# Autodesk Inventor assembly: PS20021
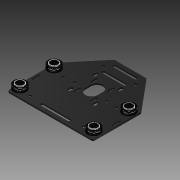
[picture p0: Inventor's stored thumbnail of the model, 180x180]
Saved by Autodesk Inventor 2014 (Build 180170000, 170)
## iProperties
Created: 2013-05-29
Part Number: PS20021
Document SubType Name: Assembly
Designer: Edward
Description: Z-Assembly Carriage
Author: Edward
Title: Z-Assembly Carriage
Subject: Shapeoko 2
## Documents named in this file (7)
- C:\Users\Edward\Documents\GitHub\Shapeoko_2\Autodesk_Inventor_Project\PS20021.iam
- C:\Users\Edward\Documents\GitHub\Shapeoko_2\Autodesk_Inventor_Project\26029-01.ipt
- C:\Users\Edward\Documents\GitHub\Shapeoko_2\Autodesk_Inventor_Project\30158-01.ipt
- C:\Users\Edward\Documents\GitHub\Shapeoko_2\Autodesk_Inventor_Project\25203-02.iam
- C:\Users\Edward\Documents\GitHub\Shapeoko_2\Autodesk_Inventor_Project\PS20004.ipt
- C:\Users\Edward\Documents\GitHub\Shapeoko_2\Autodesk_Inventor_Project\25287-02.ipt
- C:\Users\Edward\Documents\GitHub\Shapeoko_2\Autodesk_Inventor_Project\25284-02.ipt
## Components (19 placed, 6 different names)
1. 26029-01:1 — Insert:3, Insert:5, Insert:9, Mate:2, Insert:10, Mate:4, Insert:15, Insert:16
2. 30158-01:1 — Insert:10, Mate:3
3. 30158-01:2 — Mate:1, Insert:9
4. 25203-02:4 [sub-assembly] — Insert:2, Insert:4
5. 25287-02:1 — Insert:2, Insert:3
6. PS20004:2 — Insert:4
7. 25287-02:2 — Insert:11, Mate:4
8. 25284-02:2 — Insert:6
9. 25287-02:4 — Insert:16, Insert:17
10. 25287-02:5 — Insert:14, Insert:15
11. 25287-02:6 — Insert:7, Mate:2
12. 25287-02:7 — Insert:5, Insert:6
13. PS20004:3 — Insert:8, Mate:1
14. 25203-02:5 [sub-assembly] — Insert:7, Insert:8
15. PS20004:4 — Insert:12, Mate:3
16. 25203-02:6 [sub-assembly] — Insert:11, Insert:12
17. PS20004:5 — Insert:13
18. 25203-02:7 [sub-assembly] — Insert:13, Insert:14
19. 25284-02:3 — Insert:17
## Relationships (20: Insert 16, Mate 4)
- Insert:2: 25203-02:4 ↔ 25287-02:1
- Insert:3: 26029-01:1 ↔ 25287-02:1
- Insert:4: 25203-02:4 ↔ PS20004:2
- Insert:5: 26029-01:1 ↔ 25287-02:7
- Insert:6: 25284-02:2 ↔ 25287-02:7
- Insert:7: 25287-02:6 ↔ 25203-02:5
- Insert:8: PS20004:3 ↔ 25203-02:5
- Mate:1: 30158-01:2 ↔ PS20004:3
- Insert:9: 26029-01:1 ↔ 30158-01:2
- Mate:2: 26029-01:1 ↔ 25287-02:6
- Insert:10: 26029-01:1 ↔ 30158-01:1
- Insert:11: 25287-02:2 ↔ 25203-02:6
- Insert:12: PS20004:4 ↔ 25203-02:6
- Mate:3: 30158-01:1 ↔ PS20004:4
- Mate:4: 26029-01:1 ↔ 25287-02:2
- Insert:13: PS20004:5 ↔ 25203-02:7
- Insert:14: 25287-02:5 ↔ 25203-02:7
- Insert:15: 26029-01:1 ↔ 25287-02:5
- Insert:16: 26029-01:1 ↔ 25287-02:4
- Insert:17: 25287-02:4 ↔ 25284-02:3
